# Autodesk Inventor assembly: 200-50-WHEEL-CONNECTOR-20MM-ASM-01
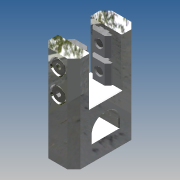
[picture p0: Inventor's stored thumbnail of the model, 180x180]
Saved by Autodesk Inventor 2018.2 (Build 222227000, 227)
## iProperties
Manager: feesmrt
Company: FRANC0R
Created: 2017-12-17
Part Number: 200-50-WHEEL-CONNECTOR-20MM-ASM-01
Document SubType Name: Assembly
Designer: feesmrt
Project: Rescue Robot
Cost Center: -
Description: Wheel Connector 20mm - ASM
Engineer: feesmrt
Authority: feesmrt
Stock Number: 200-50-WHEEL-CONNECTOR-20MM-ASM-01
Mass: 103.318 g
Surface Area: 152.396 cm^2
Volume: 30.8908 cm^3
Density: 3.34463 g/cm^3
Author: feesmrt
Title: Wheel Connector 20mm - ASM
Subject: Rescue Robot
Revision Number: 1
## Documents named in this file (6)
- D:\Programmierung\FRANC0R\CAD\02-Rocker-Bogie-Robot\200-ROCKER-BOGIE\200-50-WHEEL-CONNECTOR\200-50-WHEEL-CONNECTOR-20MM-ASM-01.iam
- D:\Programmierung\FRANC0R\CAD\02-Rocker-Bogie-Robot\200-ROCKER-BOGIE\200-50-WHEEL-CONNECTOR\200-50-WHEEL-CONNECTOR-20MM-01.ipt
- D:\Programmierung\FRANC0R\CAD\02-Rocker-Bogie-Robot\200-ROCKER-BOGIE\200-50-WHEEL-CONNECTOR\200-50-WHEEL-CONNECTOR-20MM-02.ipt
- D:\Programmierung\FRANC0R\CAD\02-Rocker-Bogie-Robot\900-COMPONENTS\900-40-SCREWS\900-40-SCREWS-DIN7984_M5x12.ipt
- D:\Programmierung\FRANC0R\CAD\02-Rocker-Bogie-Robot\900-COMPONENTS\900-50-PROFILES\900-50-PROFILES-CONN-N6xM5.ipt
- D:\Programmierung\FRANC0R\CAD\02-Rocker-Bogie-Robot\900-COMPONENTS\900-40-SCREWS\900-40-SCREWS-DIN7984_M5x10.ipt
## Components (12 placed, 5 different names)
1. 200-50-WHEEL-CONNECTOR-20MM-01:1 — Passend:5, Passend:6, Passend:7, Passend:12, Passend:13, Winkel:1, Passend:14, Passend:15, Passend:16, Passend:17, Passend:18, Passend:19, Winkel:3, Winkel:4, Passend:20, Passend:21, Passend:22, Passend:23, Passend:24, Passend:25, Passend:26, Passend:27
2. 200-50-WHEEL-CONNECTOR-20MM-02:1 — Passend:5, Passend:6, Passend:7, Passend:8, Passend:9, Passend:10, Passend:11
3. 900-40-SCREWS-DIN7984_M5x12:1 — Passend:8, Passend:9
4. 900-40-SCREWS-DIN7984_M5x12:2 — Passend:10, Passend:11
5. 900-50-PROFILES-CONN-N6xM5:1 — Passend:12, Passend:13, Winkel:1, Winkel:2
6. 900-50-PROFILES-CONN-N6xM5:2 — Passend:14, Passend:15, Winkel:2
7. 900-50-PROFILES-CONN-N6xM5:3 — Passend:16, Passend:18, Winkel:3
8. 900-50-PROFILES-CONN-N6xM5:4 — Passend:17, Passend:19, Winkel:4
9. 900-40-SCREWS-DIN7984_M5x10:1 — Passend:20, Passend:27
10. 900-40-SCREWS-DIN7984_M5x10:2 — Passend:21, Passend:26
11. 900-40-SCREWS-DIN7984_M5x10:3 — Passend:22, Passend:24
12. 900-40-SCREWS-DIN7984_M5x10:4 — Passend:23, Passend:25
## Relationships (27: Mate 23, Angle 4)
- Passend:5 [Mate]: 200-50-WHEEL-CONNECTOR-20MM-01:1 ↔ 200-50-WHEEL-CONNECTOR-20MM-02:1
- Passend:6 [Mate]: 200-50-WHEEL-CONNECTOR-20MM-01:1 ↔ 200-50-WHEEL-CONNECTOR-20MM-02:1
- Passend:7 [Mate]: 200-50-WHEEL-CONNECTOR-20MM-01:1 ↔ 200-50-WHEEL-CONNECTOR-20MM-02:1
- Passend:8 [Mate]: 200-50-WHEEL-CONNECTOR-20MM-02:1 ↔ 900-40-SCREWS-DIN7984_M5x12:1
- Passend:9 [Mate]: 200-50-WHEEL-CONNECTOR-20MM-02:1 ↔ 900-40-SCREWS-DIN7984_M5x12:1
- Passend:10 [Mate]: 200-50-WHEEL-CONNECTOR-20MM-02:1 ↔ 900-40-SCREWS-DIN7984_M5x12:2
- Passend:11 [Mate]: 200-50-WHEEL-CONNECTOR-20MM-02:1 ↔ 900-40-SCREWS-DIN7984_M5x12:2
- Passend:12 [Mate]: 200-50-WHEEL-CONNECTOR-20MM-01:1 ↔ 900-50-PROFILES-CONN-N6xM5:1
- Passend:13 [Mate] (1.5 mm): 200-50-WHEEL-CONNECTOR-20MM-01:1 ↔ 900-50-PROFILES-CONN-N6xM5:1
- Winkel:1 [Angle] (0 deg): 200-50-WHEEL-CONNECTOR-20MM-01:1 ↔ 900-50-PROFILES-CONN-N6xM5:1
- Passend:14 [Mate]: 200-50-WHEEL-CONNECTOR-20MM-01:1 ↔ 900-50-PROFILES-CONN-N6xM5:2
- Passend:15 [Mate] (1.5 mm): 200-50-WHEEL-CONNECTOR-20MM-01:1 ↔ 900-50-PROFILES-CONN-N6xM5:2
- Winkel:2 [Angle] (0 deg): 900-50-PROFILES-CONN-N6xM5:1 ↔ 900-50-PROFILES-CONN-N6xM5:2
- Passend:16 [Mate]: 200-50-WHEEL-CONNECTOR-20MM-01:1 ↔ 900-50-PROFILES-CONN-N6xM5:3
- Passend:17 [Mate]: 200-50-WHEEL-CONNECTOR-20MM-01:1 ↔ 900-50-PROFILES-CONN-N6xM5:4
- Passend:18 [Mate] (1.5 mm): 200-50-WHEEL-CONNECTOR-20MM-01:1 ↔ 900-50-PROFILES-CONN-N6xM5:3
- Passend:19 [Mate] (1.5 mm): 200-50-WHEEL-CONNECTOR-20MM-01:1 ↔ 900-50-PROFILES-CONN-N6xM5:4
- Winkel:3 [Angle] (0 deg): 200-50-WHEEL-CONNECTOR-20MM-01:1 ↔ 900-50-PROFILES-CONN-N6xM5:3
- Winkel:4 [Angle] (0 deg): 200-50-WHEEL-CONNECTOR-20MM-01:1 ↔ 900-50-PROFILES-CONN-N6xM5:4
- Passend:20 [Mate]: 200-50-WHEEL-CONNECTOR-20MM-01:1 ↔ 900-40-SCREWS-DIN7984_M5x10:1
- Passend:21 [Mate]: 200-50-WHEEL-CONNECTOR-20MM-01:1 ↔ 900-40-SCREWS-DIN7984_M5x10:2
- Passend:22 [Mate]: 200-50-WHEEL-CONNECTOR-20MM-01:1 ↔ 900-40-SCREWS-DIN7984_M5x10:3
- Passend:23 [Mate]: 200-50-WHEEL-CONNECTOR-20MM-01:1 ↔ 900-40-SCREWS-DIN7984_M5x10:4
- Passend:24 [Mate]: 200-50-WHEEL-CONNECTOR-20MM-01:1 ↔ 900-40-SCREWS-DIN7984_M5x10:3
- Passend:25 [Mate]: 200-50-WHEEL-CONNECTOR-20MM-01:1 ↔ 900-40-SCREWS-DIN7984_M5x10:4
- Passend:26 [Mate]: 200-50-WHEEL-CONNECTOR-20MM-01:1 ↔ 900-40-SCREWS-DIN7984_M5x10:2
- Passend:27 [Mate]: 200-50-WHEEL-CONNECTOR-20MM-01:1 ↔ 900-40-SCREWS-DIN7984_M5x10:1
